# Autodesk Inventor assembly: rod_v4
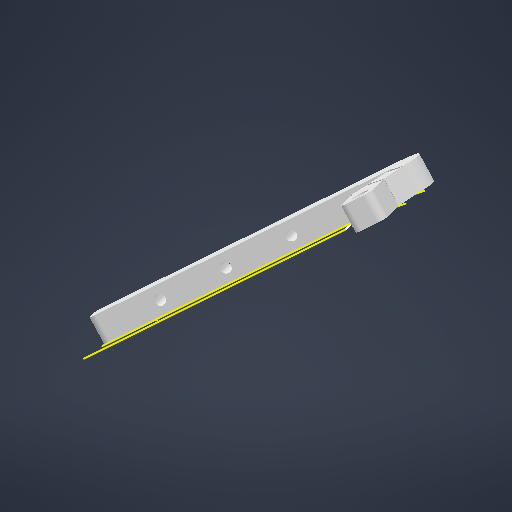
[picture p0: Inventor's stored thumbnail of the model, 512x512]
Saved by Autodesk Inventor 2026.2 (Build 302298000, 298)
## iProperties
Created: 2025-12-17
Part Number: rod_v4
Document SubType Name: Assembly
Designer: Thoma
Author: Thoma
## Documents named in this file (4)
- C:\Users\Thoma\OneDrive\Desktop\Inventor\Quarter_Open\Version_2_Cone\rod_v4.iam
- C:\Users\Thoma\OneDrive\Desktop\Inventor\Quarter_Open\Version_2_Cone\rod_v2.5.ipt
- C:\Users\Thoma\OneDrive\Desktop\Inventor\Quarter_Open\Version_2_Cone\rod_v2.6.ipt
- C:\Users\Thoma\OneDrive\Desktop\Inventor\Quarter_Open\Version_2_Cone\rod_v2.ipt
## Components (3 placed, 3 different names)
1. rod_v2.5:1 — Mate:3, Flush:2, Mate:4
2. rod_v2.6:1 — Flush:1, Mate:3, Flush:2, Mate:4, Mate:5, Mate:6
3. rod_v2:1 — Flush:1, Mate:5, Mate:6
## Relationships (6: Mate 4, Flush 2)
- Flush:1: rod_v2.6:1 ↔ rod_v2:1
- Mate:3: rod_v2.5:1 ↔ rod_v2.6:1
- Flush:2: rod_v2.5:1 ↔ rod_v2.6:1
- Mate:4: rod_v2.5:1 ↔ rod_v2.6:1
- Mate:5: rod_v2.6:1 ↔ rod_v2:1
- Mate:6: rod_v2.6:1 ↔ rod_v2:1
